# Autodesk Inventor assembly: s-assy-sorter_plate
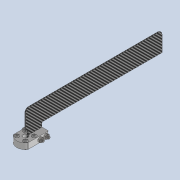
[picture p0: Inventor's stored thumbnail of the model, 180x180]
Saved by Autodesk Inventor 2022 (Build 260153000, 153)
## iProperties
Created: 2021-08-27
Part Number: s-assy-sorter_plate
Document SubType Name: Assembly
Designer: Yuta Kage
Author: Yuta Kage
## Documents named in this file (6)
- C:\Users\yuta0\Desktop\catchrobo_hardware-main\catchrobo_hardware-main\assy-shooter\s-assy-sorter_plate.iam
- C:\Users\yuta0\Desktop\catchrobo_hardware-main\catchrobo_hardware-main\assy-shooter\shooter_base3.ipt
- C:\Users\yuta0\Desktop\catchrobo_hardware-main\catchrobo_hardware-main\assy-shooter\CB3-25.ipt
- C:\Users\yuta0\Desktop\catchrobo_hardware-main\catchrobo_hardware-main\assy-shooter\LBNR3.ipt
- C:\Users\yuta0\Desktop\catchrobo_hardware-main\catchrobo_hardware-main\assy-shooter\shooter_carbon_plate2.ipt
- C:\Users\yuta0\Desktop\catchrobo_hardware-main\catchrobo_hardware-main\assy-shooter\CBSTSR3-10.ipt
## Components (10 placed, 5 different names)
1. shooter_base3:1 — メイト:77, メイト:78, メイト:79, メイト:80, メイト:81, メイト:83, メイト:84, フラッシュ:1, フラッシュ:2, メイト:85, メイト:86
2. shooter_carbon_plate2:1 — メイト:77, メイト:78, メイト:79
3. LBNR3:1 — メイト:82, メイト:83
4. CB3-25:1 — メイト:80, メイト:81, メイト:82
5. LBNR3:2
6. CB3-25:2
7. CBSTSR3-10:2 — メイト:85, メイト:86
8. CBSTSR3-10:3
9. CBSTSR3-10:4
10. CBSTSR3-10:5
## Component patterns: (2 elements, first: LBNR3:1 + CB3-25:1), (4 elements, first: CBSTSR3-10:2)
## Relationships (12: Mate 10, Flush 2)
- メイト:77 [Mate]: shooter_base3:1 ↔ shooter_carbon_plate2:1
- メイト:78 [Mate]: shooter_base3:1 ↔ shooter_carbon_plate2:1
- メイト:79 [Mate]: shooter_base3:1 ↔ shooter_carbon_plate2:1
- メイト:80 [Mate]: shooter_base3:1 ↔ CB3-25:1
- メイト:81 [Mate]: shooter_base3:1 ↔ CB3-25:1
- メイト:82 [Mate]: LBNR3:1 ↔ CB3-25:1
- メイト:83 [Mate]: shooter_base3:1 ↔ LBNR3:1
- メイト:84 [Mate]: shooter_base3:1
- フラッシュ:1 [Flush]: shooter_base3:1
- フラッシュ:2 [Flush]: shooter_base3:1
- メイト:85 [Mate]: shooter_base3:1 ↔ CBSTSR3-10:2
- メイト:86 [Mate]: shooter_base3:1 ↔ CBSTSR3-10:2
